# Autodesk Inventor assembly: Axle-Assembly
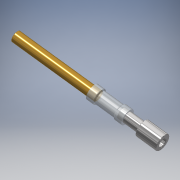
[picture p0: Inventor's stored thumbnail of the model, 180x180]
Saved by Autodesk Inventor 2016 (Build 200138000, 138)
## iProperties
Created: 2015-05-19
Part Number: Axle-Assembly
Document SubType Name: Assembly
Designer: jonathan
Mass: 3.28411 g
Surface Area: 30.922 cm^2
Volume: 3.28411 cm^3
Density: 1 g/cm^3
Author: jonathan
## Documents named in this file (4)
- C:\Users\jonathan\Desktop\CLEAN COPIES\DC Motor Test Stand\Inventor\Axle Assembly.iam
- C:\Users\jonathan\Desktop\CLEAN COPIES\DC Motor Test Stand\Inventor\Motor Adapter.ipt
- C:\Users\jonathan\Desktop\CLEAN COPIES\DC Motor Test Stand\Inventor\Axle Brass.ipt
- C:\Users\jonathan\Desktop\CLEAN COPIES\DC Motor Test Stand\Inventor\Axle Connector.ipt
## Components (3 placed, 3 different names)
1. Motor Adapter:1 — Mate:1, Mate:3, Mate:4
2. Axle Brass:1 — Mate:5, Mate:6
3. Axle Connector:1 — Mate:1, Mate:3, Mate:4, Mate:5, Mate:6
## Relationships (5: Mate 5)
- Mate:1: Motor Adapter:1 ↔ Axle Connector:1
- Mate:3: Motor Adapter:1 ↔ Axle Connector:1
- Mate:4 (-3.81 mm): Motor Adapter:1 ↔ Axle Connector:1
- Mate:5: Axle Brass:1 ↔ Axle Connector:1
- Mate:6 (-3.81 mm): Axle Brass:1 ↔ Axle Connector:1
